# Autodesk Inventor assembly: bigLipo
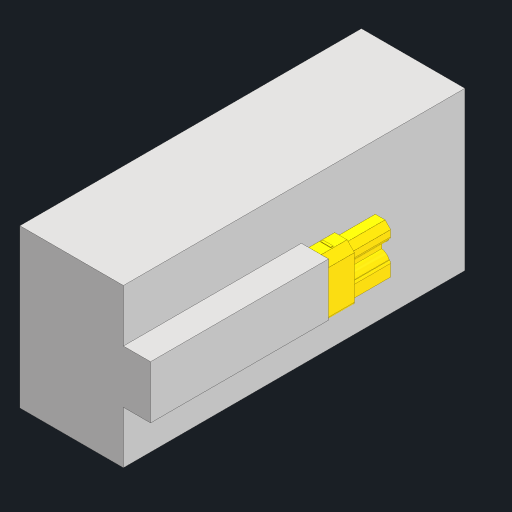
[picture p0: Inventor's stored thumbnail of the model, 512x512]
Saved by Autodesk Inventor 2023 (Build 270158000, 158)
## iProperties
Created: 2024-04-13
Part Number: bigLipo
Document SubType Name: Assembly
Designer: szymo
Mass: 65 g
Surface Area: 99.0233 cm^2
Volume: 42.7256 cm^3
Density: 1.52134 g/cm^3
Author: szymo
## Documents named in this file (3)
- C:\zRozne\roboilo\robots\wafel\3d_parts\bigLipo.iam
- C:\zRozne\roboilo\robots\wafel\3d_parts\xt30.ipt
- C:\zRozne\roboilo\robots\wafel\3d_parts\lipo3s650.ipt
## Components (2 placed, 2 different names)
1. xt30:1 — Mate:1, Flush:1, Flush:2
2. lipo3s650:1 — Mate:1, Flush:1, Flush:2
## Relationships (3: Flush 2, Mate 1)
- Mate:1: xt30:1 ↔ lipo3s650:1
- Flush:1 (19 mm): xt30:1 ↔ lipo3s650:1
- Flush:2 (-10.125 mm): xt30:1 ↔ lipo3s650:1
